# Autodesk Inventor assembly: Connessione B
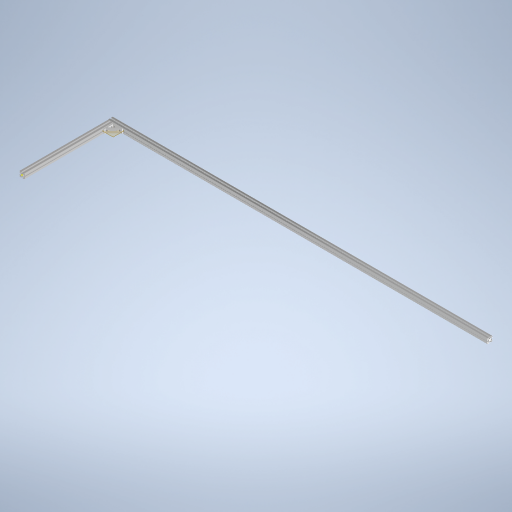
[picture p0: Inventor's stored thumbnail of the model, 512x512]
Saved by Autodesk Inventor 2023 (Build 270158000, 158)
## iProperties
Created: 2022-01-26
Part Number: Connessione B
Document SubType Name: Assembly
Designer: matte
Author: matte
## Documents named in this file (6)
- C:\Users\matte\Documents\GitHub\MDM-CyberOrto-CAD\Esplosi\Connessione B.iam
- C:\Users\matte\Documents\GitHub\MDM-CyberOrto-CAD\Parker components\03-Brackets_Gussets_Plates\09-Machined Gussets\20-102.ipt
- C:\Users\matte\Documents\GitHub\MDM-CyberOrto-CAD\Parker components\02-Fasteners\10-Standard T-Nuts\20-050.ipt
- C:\Users\matte\Documents\GitHub\MDM-CyberOrto-CAD\Parker components\02-Fasteners\16-Screws\01-Metric Screws\01-Button Head\24-118-8.ipt
- C:\Users\matte\Documents\GitHub\MDM-CyberOrto-CAD\Pezzi singoli\Supporto SX.ipt
- C:\Users\matte\Documents\GitHub\MDM-CyberOrto-CAD\Pezzi singoli\10-040.ipt
## Components (9 placed, 5 different names)
1. Supporto SX:2
2. 20-102:2
3. 20-050:3
4. 20-050:4
5. 24-118-8:5
6. 24-118-8:6
7. 24-118-8:7
8. 24-118-8:8
9. 10-040:2
## Relationships (20: Mate 17, Flush 3)
- [Mate]: 20-102:2 ↔ 10-040:2
- [Mate]: Supporto SX:2 ↔ 20-102:2
- [Flush]: Supporto SX:2 ↔ 20-102:2
- [Mate]: Supporto SX:2 ↔ 20-050:3
- [Mate]: 20-102:2 ↔ 20-050:3
- [Mate]: 20-102:2 ↔ 20-050:3
- [Mate]: 20-050:4 ↔ 10-040:2
- [Mate]: 20-102:2 ↔ 20-050:4
- [Mate]: 20-102:2 ↔ 20-050:4
- [Mate]: 20-102:2 ↔ 24-118-8:5
- [Mate]: 20-102:2 ↔ 24-118-8:5
- [Mate]: 20-102:2 ↔ 24-118-8:6
- [Mate]: 20-102:2 ↔ 24-118-8:6
- [Mate]: 20-102:2 ↔ 24-118-8:7
- [Mate]: 20-102:2 ↔ 24-118-8:7
- [Mate]: 20-102:2 ↔ 24-118-8:8
- [Mate]: 20-102:2 ↔ 24-118-8:8
- [Flush]: Supporto SX:2 ↔ 10-040:2
- [Mate]: Supporto SX:2 ↔ 10-040:2
- [Flush]: Supporto SX:2 ↔ 10-040:2
## Named parameters: d51_d15 = 0 mm, d52_d16 = 0 mm, d54_d18 = 0 mm, d55_d19 = 0 mm, d56_d20 = 0 mm, d57_d21 = 0 mm, d58_d24 = 0 mm, d59_d25 = 0 mm, d60_d26 = 0 mm, d61_d27 = 0 mm, d62_d28 = 0 mm, d63_d29 = 0 mm
